# Autodesk Inventor assembly: ASY PNS 1100 left module
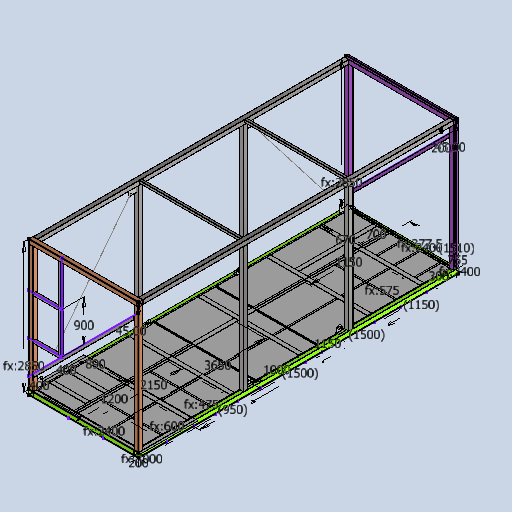
[picture p0: Inventor's stored thumbnail of the model, 512x512]
Saved by Autodesk Inventor 2025 (Build 290162010, 162A)
## iProperties
Created: 2025-03-25
Part Number: ASY PNS 1100 left module
Document SubType Name: Assembly
Designer: user
Mass: 1.00117e+06 g
Surface Area: 692723 cm^2
Volume: 127418 cm^3
Density: 7.85736 g/cm^3
Author: user
## Documents named in this file (9)
- C:\Users\user\YandexDisk-badmisterfox\home pc\Inventor\PNS2-Panaevsk\ASY PNS 1100 left module.iam
- C:\Users\user\YandexDisk-badmisterfox\home pc\Inventor\PNS2-Panaevsk\ASY PNS 1110 frame left floor.iam
- C:\Users\user\YandexDisk-badmisterfox\home pc\Inventor\PNS2-Panaevsk\ASY PNS 1120 frame featheredge.iam
- C:\Users\user\YandexDisk-badmisterfox\home pc\Inventor\PNS2-Panaevsk\ASY PNS 1130 frame featheredge.iam
- C:\Users\user\YandexDisk-badmisterfox\home pc\Inventor\PNS2-Panaevsk\PNS-0261 Upper beam.ipt
- C:\Users\user\YandexDisk-badmisterfox\home pc\Inventor\PNS2-Panaevsk\PNS-0262 middle pillar.ipt
- C:\Users\user\YandexDisk-badmisterfox\home pc\Inventor\PNS2-Panaevsk\PNS-071 stretch ring.ipt
- C:\Users\user\YandexDisk-badmisterfox\home pc\Inventor\PNS2-Panaevsk\PNS-0310 strench.ipt
- C:\Users\user\YandexDisk-badmisterfox\home pc\Inventor\PNS2-Panaevsk\PNS-0262 cross beam.ipt
## Components (17 placed, 8 different names)
1. ASY PNS-0110 frame left floor:1 [sub-assembly]
2. ASY PNS-0250 frame featheredge 0260:1 [sub-assembly] — Rigid:3, Rigid:4, Rigid:6, Rigid:7
3. ASY PNS-0250 frame featheredge 0270:1 [sub-assembly] — Rigid:5, Rigid:8
4. PNS-0261 Upper beam:1 — Rigid:3, Mate:4, Flush:2, Mate:5, Flush:3
5. PNS-0261 Upper beam:2 — Rigid:4
6. PNS-0262 middle pillar:1 — Rigid:5, Flush:4
7. PNS-0262 middle pillar:2 — Rigid:8
8. PNS-0262 middle pillar:3 — Rigid:7
9. PNS-0262 middle pillar:4 — Rigid:6, Flush:5
10. PNS-071 stretch ring:1 — Mate:1, Flush:1
11. PNS-071 stretch ring:2
12. PNS-0310 strench:1 — Mate:1, Flush:1
13. PNS-071 stretch ring:3 — Mate:2, Mate:3
14. PNS-071 stretch ring:4
15. PNS-0310 strench:2 — Mate:2, Mate:3
16. PNS-0262 cross beam:1 — Mate:5, Flush:3, Flush:4
17. PNS-0262 cross beam:2 — Mate:4, Flush:2, Flush:5
## Relationships (18: WeldJoint 8, Mate 5, Flush 5)
- [WeldJoint]: ASY PNS-0110 frame left floor:1 ↔ ASY PNS-0250 frame featheredge 0260:1
- [WeldJoint]: ASY PNS-0110 frame left floor:1 ↔ ASY PNS-0250 frame featheredge 0270:1
- Rigid:3 [WeldJoint] (-100 mm): ASY PNS-0250 frame featheredge 0260:1 ↔ PNS-0261 Upper beam:1
- Rigid:4 [WeldJoint] (-100 mm): ASY PNS-0250 frame featheredge 0260:1 ↔ PNS-0261 Upper beam:2
- Rigid:5 [WeldJoint] (2200 mm): ASY PNS-0250 frame featheredge 0270:1 ↔ PNS-0262 middle pillar:1
- Rigid:6 [WeldJoint] (2200 mm): ASY PNS-0250 frame featheredge 0260:1 ↔ PNS-0262 middle pillar:4
- Rigid:7 [WeldJoint] (2200 mm): ASY PNS-0250 frame featheredge 0260:1 ↔ PNS-0262 middle pillar:3
- Rigid:8 [WeldJoint] (2200 mm): ASY PNS-0250 frame featheredge 0270:1 ↔ PNS-0262 middle pillar:2
- Mate:1: PNS-071 stretch ring:1 ↔ PNS-0310 strench:1
- Flush:1: PNS-071 stretch ring:1 ↔ PNS-0310 strench:1
- Mate:2: PNS-071 stretch ring:3 ↔ PNS-0310 strench:2
- Mate:3: PNS-071 stretch ring:3 ↔ PNS-0310 strench:2
- Mate:4: PNS-0261 Upper beam:1 ↔ PNS-0262 cross beam:2
- Flush:2: PNS-0261 Upper beam:1 ↔ PNS-0262 cross beam:2
- Mate:5: PNS-0261 Upper beam:1 ↔ PNS-0262 cross beam:1
- Flush:3: PNS-0261 Upper beam:1 ↔ PNS-0262 cross beam:1
- Flush:4 (20 mm): PNS-0262 middle pillar:1 ↔ PNS-0262 cross beam:1
- Flush:5 (20 mm): PNS-0262 middle pillar:4 ↔ PNS-0262 cross beam:2
